# Autodesk Inventor assembly: tensioner2
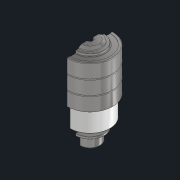
[picture p0: Inventor's stored thumbnail of the model, 180x180]
Saved by Autodesk Inventor 2021 (Build 250183000, 183)
## iProperties
Created: 2021-07-18
Part Number: tensioner2
Document SubType Name: Assembly
Designer: yuta0
Mass: 26.9565 g
Surface Area: 38.6954 cm^2
Volume: 3.73485 cm^3
Density: 7.21757 g/cm^3
Author: yuta0
## Documents named in this file (7)
- C:\Users\yuta0\Documents\GitHub\catchrobo_hardware\catchrobo_robot\tensioner2.iam
- C:\Users\yuta0\Documents\GitHub\catchrobo_hardware\catchrobo_robot\B688ZZ.ipt
- C:\Users\yuta0\Documents\GitHub\catchrobo_hardware\catchrobo_robot\WSJ-STN-M4.ipt
- C:\Users\yuta0\Documents\GitHub\catchrobo_hardware\catchrobo_robot\CBSTSR4-6.ipt
- C:\Users\yuta0\Documents\GitHub\catchrobo_hardware\catchrobo_robot\base40.ipt
- C:\Users\yuta0\Documents\GitHub\catchrobo_hardware\catchrobo_robot\ARF-420E.ipt
- C:\Users\yuta0\Documents\GitHub\catchrobo_hardware\catchrobo_robot\CB4-10.ipt
## Components (9 placed, 6 different names)
1. ARF-420E:1 — メイト:1, メイト:7, メイト:8, メイト:14, メイト:16, メイト:17
2. CB4-10:1 — メイト:20, メイト:21
3. WSJ-STN-M4:1 — メイト:7, メイト:8, メイト:15
4. WSJ-STN-M4:2 — メイト:18, メイト:19, メイト:20, メイト:21
5. CBSTSR4-6:1 — メイト:14, メイト:15
6. base40:1 — メイト:16, メイト:17, メイト:18, メイト:19, メイト:22
7. B688ZZ:1 — メイト:1, メイト:22
8. B688ZZ:2
9. B688ZZ:3
## Component patterns: (3 elements, first: B688ZZ:1)
## Relationships (12: Mate 12)
- メイト:1 [Mate]: ARF-420E:1 ↔ B688ZZ:1
- メイト:7 [Mate]: ARF-420E:1 ↔ WSJ-STN-M4:1
- メイト:8 [Mate]: ARF-420E:1 ↔ WSJ-STN-M4:1
- メイト:14 [Mate]: ARF-420E:1 ↔ CBSTSR4-6:1
- メイト:15 [Mate]: WSJ-STN-M4:1 ↔ CBSTSR4-6:1
- メイト:16 [Mate]: ARF-420E:1 ↔ base40:1
- メイト:17 [Mate]: ARF-420E:1 ↔ base40:1
- メイト:18 [Mate] (2 mm): WSJ-STN-M4:2 ↔ base40:1
- メイト:19 [Mate]: WSJ-STN-M4:2 ↔ base40:1
- メイト:20 [Mate]: CB4-10:1 ↔ WSJ-STN-M4:2
- メイト:21 [Mate]: CB4-10:1 ↔ WSJ-STN-M4:2
- メイト:22 [Mate]: base40:1 ↔ B688ZZ:1
